# Autodesk Inventor assembly: Z Extrusion Left
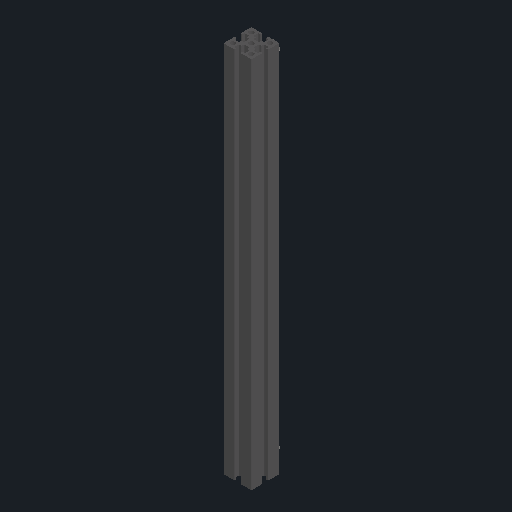
[picture p0: Inventor's stored thumbnail of the model, 512x512]
Saved by Autodesk Inventor 2025.1 (Build 291241020, 241B)
## iProperties
Created: 2025-05-11
Part Number: Z Extrusion Left
Document SubType Name: Assembly
Designer: Joshua Eah
Author: Joshua Eah
## Documents named in this file (4)
- C:\Users\Joshua Eah\Documents\Voron 0.2\CAD\Master Assembly\Z Extrusion Left.iam
- C:\Users\Joshua Eah\Documents\Voron 0.2\CAD\Master Assembly\Frame\Parts\Extrusions\1515_200mm - C.ipt
- C:\Users\Joshua Eah\Documents\Voron 0.2\CAD\Master Assembly\Hardware\M3x6 BHCS.ipt
- C:\Users\Joshua Eah\Documents\Voron 0.2\CAD\Master Assembly\Hardware\M3 Hexnut.ipt
## Components (5 placed, 3 different names)
1. 1515_200mm - C:3
2. M3x6 BHCS:1
3. M3x6 BHCS:2
4. M3 Hexnut:6
5. M3 Hexnut:7
## Relationships (6: Mate 4, Insert 2)
- [Mate]: 1515_200mm - C:3 ↔ M3x6 BHCS:1
- [Mate]: 1515_200mm - C:3 ↔ M3x6 BHCS:1
- [Mate]: 1515_200mm - C:3 ↔ M3x6 BHCS:2
- [Mate]: 1515_200mm - C:3 ↔ M3x6 BHCS:2
- [Insert]: M3x6 BHCS:1 ↔ M3 Hexnut:7
- [Insert]: M3x6 BHCS:2 ↔ M3 Hexnut:6
## Named parameters: d0_d2 = 0 mm, d1_d3 = 0 mm
